# Autodesk Inventor assembly: Ender-3
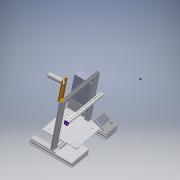
[picture p0: Inventor's stored thumbnail of the model, 180x180]
Saved by Autodesk Inventor 2017 (Build 210142000, 142)
## iProperties
Created: 2018-07-04
Part Number: Ender-3
Document SubType Name: Assembly
Designer: UnKnoWn
Author: UnKnoWn
## Documents named in this file (12)
- I:\3d Printer stuff\Ender 3\Ender3 working files\Ender-3.iam
- I:\3d Printer stuff\Ender 3\Ender3 working files\Ender-3 Mechanical\STP\2020-2 profile.ipt
- I:\3d Printer stuff\Ender 3\Ender3 working files\Ender-3 Mechanical\STP\2040 profile.ipt
- I:\3d Printer stuff\Ender 3\Ender3 working files\Ender-3 Mechanical\STP\4040 profile.ipt
- I:\3d Printer stuff\Ender 3\Ender3 working files\Ender-3 Mechanical\STP\top_rail.ipt
- I:\3d Printer stuff\Ender 3\Ender3 working files\Ender-3 Mechanical\STP\powersupply assm.iam
- I:\3d Printer stuff\Ender 3\Ender3 working files\Ender-3 Mechanical\STP\Support frame.ipt
- I:\3d Printer stuff\Ender 3\Ender3 working files\Ender-3 Mechanical\STP\Support tube.ipt
- I:\3d Printer stuff\Ender 3\Ender3 working files\Ender-3 Mechanical\STP\Eccentric column.ipt
- I:\3d Printer stuff\Ender 3\Ender3 working files\Ender-3 Mechanical\STP\Hot bed.ipt
- I:\3d Printer stuff\Ender 3\Ender3 working files\Ender-3 Mechanical\STP\controlbox.iam
- I:\3d Printer stuff\Ender 3\Ender3 working files\Ender-3 Mechanical\STP\lcdAssembly.iam
## Components (14 placed, 11 different names)
1. 2020-2 profile:1
2. 2040 profile:1 — Mate:7, Mate:8, Mate:9, Mate:14, Mate:15
3. 4040 profile:1 — Mate:4, Mate:5, Mate:6, Mate:7, Mate:8, Mate:9
4. 4040 profile:2 — Mate:1, Mate:2, Mate:3, Mate:11, Mate:12, Mate:13
5. 4040 profile:3 — Mate:1, Mate:2, Mate:3, Mate:4, Mate:5, Mate:6
6. 2040 profile:2 — Mate:11, Mate:12, Mate:13, Mate:16
7. top_rail:1 — Mate:14, Mate:15, Mate:16
8. powersupply assm:1 [sub-assembly]
9. Support frame:1
10. Support tube:1
11. Eccentric column:1
12. Hot bed:1
13. controlbox:1 [sub-assembly]
14. lcdAssembly:1 [sub-assembly]
## Relationships (15: Mate 15)
- Mate:1: 4040 profile:2 ↔ 4040 profile:3
- Mate:2: 4040 profile:2 ↔ 4040 profile:3
- Mate:3: 4040 profile:2 ↔ 4040 profile:3
- Mate:4: 4040 profile:1 ↔ 4040 profile:3
- Mate:5: 4040 profile:1 ↔ 4040 profile:3
- Mate:6: 4040 profile:1 ↔ 4040 profile:3
- Mate:7: 2040 profile:1 ↔ 4040 profile:1
- Mate:8: 2040 profile:1 ↔ 4040 profile:1
- Mate:9: 2040 profile:1 ↔ 4040 profile:1
- Mate:11: 4040 profile:2 ↔ 2040 profile:2
- Mate:12: 4040 profile:2 ↔ 2040 profile:2
- Mate:13: 4040 profile:2 ↔ 2040 profile:2
- Mate:14: 2040 profile:1 ↔ top_rail:1
- Mate:15: 2040 profile:1 ↔ top_rail:1
- Mate:16: 2040 profile:2 ↔ top_rail:1
